# Autodesk Inventor assembly: Engine Assembly
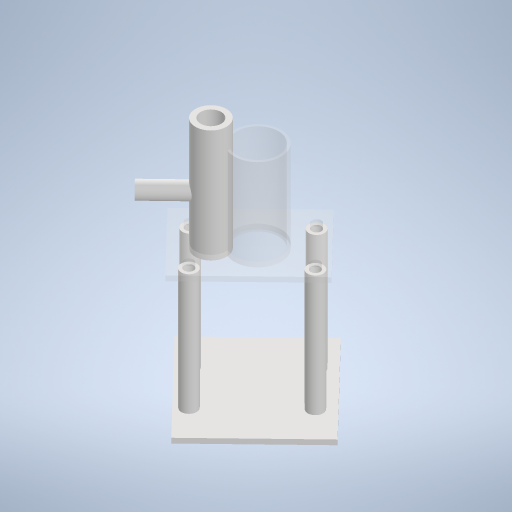
[picture p0: Inventor's stored thumbnail of the model, 512x512]
Saved by Autodesk Inventor 2023 (Build 270158000, 158)
## iProperties
Created: 2023-02-13
Part Number: Engine Assembly
Document SubType Name: Assembly
Designer: tommy
Author: tommy
## Documents named in this file (4)
- C:\Users\tommy\Documents\Repositories\Steam-Engine\Les Proper Steam Engine\CAD\Engine Assembly.iam
- C:\Users\tommy\Documents\Repositories\Steam-Engine\Les Proper Steam Engine\CAD\Base Bottom.ipt
- C:\Users\tommy\Documents\Repositories\Steam-Engine\Les Proper Steam Engine\CAD\Frame Post.ipt
- C:\Users\tommy\Documents\Repositories\Steam-Engine\Les Proper Steam Engine\CAD\Cylinder Assembly.iam
## Components (6 placed, 3 different names)
1. Base Bottom:1 — Mate:9, Mate:10, Mate:11, Mate:12, Mate:13, Mate:14, Mate:15, Mate:16, Mate:17
2. Frame Post:1 — Mate:14, Mate:16
3. Frame Post:2 — Mate:9, Mate:10, Mate:18
4. Frame Post:3 — Mate:11, Mate:13, Mate:17, Mate:20
5. Frame Post:4 — Mate:12, Mate:15, Mate:19
6. Cylinder Assembly:1 [sub-assembly] — Mate:18, Mate:19, Mate:20
## Relationships (12: Mate 12)
- Mate:9: Base Bottom:1 ↔ Frame Post:2
- Mate:10: Base Bottom:1 ↔ Frame Post:2
- Mate:11: Base Bottom:1 ↔ Frame Post:3
- Mate:12: Base Bottom:1 ↔ Frame Post:4
- Mate:13: Base Bottom:1 ↔ Frame Post:3
- Mate:14: Base Bottom:1 ↔ Frame Post:1
- Mate:15: Base Bottom:1 ↔ Frame Post:4
- Mate:16: Base Bottom:1 ↔ Frame Post:1
- Mate:17: Base Bottom:1 ↔ Frame Post:3
- Mate:18: Frame Post:2 ↔ Cylinder Assembly:1
- Mate:19: Frame Post:4 ↔ Cylinder Assembly:1
- Mate:20: Frame Post:3 ↔ Cylinder Assembly:1
